# Autodesk Inventor assembly: 000 ASY GBK Gubkinskiy
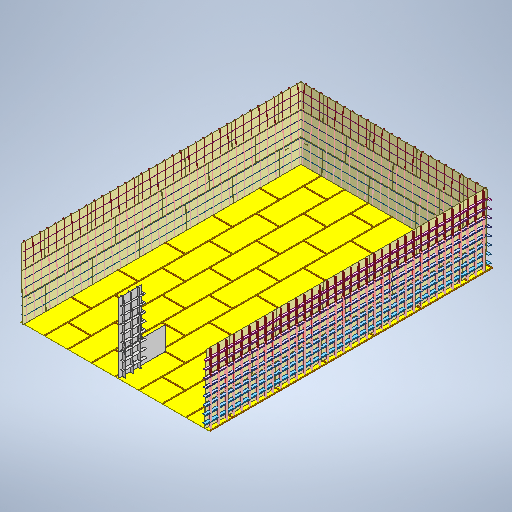
[picture p0: Inventor's stored thumbnail of the model, 512x512]
Saved by Autodesk Inventor 2026.2 (Build 302298000, 298)
## iProperties
Created: 2026-04-17
Part Number: 000 ASY GBK Gubkinskiy
Document SubType Name: Assembly
Designer: admin
Mass: 2.02017e+07 g
Surface Area: 1.30705e+07 cm^2
Volume: 2.57346e+06 cm^3
Density: 7.85 g/cm^3
Author: admin
## Documents named in this file (11)
- C:\Users\admin\Documents\Inventor\GBK-Gubkinskiy\000 ASY GBK Gubkinskiy.iam
- C:\Users\admin\Documents\Inventor\GBK-Gubkinskiy\GBK bottom.ipt
- C:\Users\admin\Documents\Inventor\GBK-Gubkinskiy\GBK dummy wall 1.ipt
- C:\Users\admin\Documents\Inventor\GBK-Gubkinskiy\GBK dummy wall 4.ipt
- C:\Users\admin\Documents\Inventor\GBK-Gubkinskiy\GBK overall model.ipt
- C:\Users\admin\Documents\Inventor\GBK-Gubkinskiy\0401 ASY GBK wall shield Center 1.iam
- C:\Users\admin\Documents\Inventor\GBK-Gubkinskiy\0701 ASY GBK wall shield Center 4.iam
- C:\Users\admin\Documents\Inventor\GBK-Gubkinskiy\01001 ASY GBK wall shield Center 10.iam
- C:\Users\admin\Documents\Inventor\GBK-Gubkinskiy\ASY GBK правая стенка.iam
- C:\Users\admin\Documents\Inventor\GBK-Gubkinskiy\ASY GBK предварительная торцевая.iam
- C:\Users\admin\Documents\Inventor\GBK-Gubkinskiy\090 ASY bottom.iam
## Components (13 placed, 10 different names)
1. GBK bottom.ipt:1 — Mate:10, Mate:11, Mate:12, Mate:13, Mate:14, Rigid:1, Flush:4, Flush:6, Flush:7, Flush:8
2. GBK dummy wall 1.ipt:1 — Mate:10
3. GBK dummy wall 1.ipt:2 — Mate:11, Mate:12
4. GBK dummy wall 4.ipt:1 — Mate:13, Mate:14
5. GBK overall model:1 — Rigid:1
6. ASY GBK правая стенка:1 [sub-assembly]
7. ASY GBK предварительная торцевая:1 [sub-assembly]
8. ASY GBK предварительная торцевая:2 [sub-assembly] — Mate:17, Flush:4
9. ASY GBK правая стенка:2 [sub-assembly] — Flush:5, Flush:6
10. 0701 ASY GBK wall shield Center 4:1 [sub-assembly] — Rigid:2, Rigid:3
11. 01001 ASY GBK wall shield Center 10:1 [sub-assembly] — Rigid:3
12. 0401 ASY GBK wall shield Center 1:1 [sub-assembly] — Rigid:2, Mate:18, Flush:7
13. 090 ASY bottom:1 [sub-assembly] — Mate:19, Flush:8
## Relationships (20: Mate 10, Flush 7, WeldJoint 3)
- [Flush]: GBK bottom.ipt:1 ↔ ASY GBK правая стенка:1
- [Mate]: GBK bottom.ipt:1 ↔ ASY GBK правая стенка:1
- Mate:10: GBK bottom.ipt:1 ↔ GBK dummy wall 1.ipt:1
- Mate:11: GBK bottom.ipt:1 ↔ GBK dummy wall 1.ipt:2
- Mate:12: GBK bottom.ipt:1 ↔ GBK dummy wall 1.ipt:2
- Mate:13: GBK bottom.ipt:1 ↔ GBK dummy wall 4.ipt:1
- Mate:14: GBK bottom.ipt:1 ↔ GBK dummy wall 4.ipt:1
- Rigid:1 [WeldJoint]: GBK bottom.ipt:1 ↔ GBK overall model:1
- [Mate]: ASY GBK предварительная торцевая:1
- [Flush]: GBK bottom.ipt:1 ↔ ASY GBK предварительная торцевая:1
- Mate:17: ASY GBK предварительная торцевая:2
- Flush:4: GBK bottom.ipt:1 ↔ ASY GBK предварительная торцевая:2
- Flush:5: ASY GBK правая стенка:2
- Flush:6: GBK bottom.ipt:1 ↔ ASY GBK правая стенка:2
- Rigid:2 [WeldJoint]: 0701 ASY GBK wall shield Center 4:1 ↔ 0401 ASY GBK wall shield Center 1:1
- Rigid:3 [WeldJoint]: 0701 ASY GBK wall shield Center 4:1 ↔ 01001 ASY GBK wall shield Center 10:1
- Mate:18: 0401 ASY GBK wall shield Center 1:1
- Flush:7: GBK bottom.ipt:1 ↔ 0401 ASY GBK wall shield Center 1:1
- Mate:19: 090 ASY bottom:1
- Flush:8: GBK bottom.ipt:1 ↔ 090 ASY bottom:1
## Named parameters: Зазор_по_горизонту = 1 mm, d120_Зазор_по_горизонту = 1 mm, d141_Зазор_по_горизонту = 1 mm, d159_d141_Зазор_по_горизонту = 1 mm, d175_d141_Зазор_по_горизонту = 1 mm
